# Autodesk Inventor assembly: 044-DPK
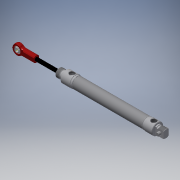
[picture p0: Inventor's stored thumbnail of the model, 180x180]
Saved by Autodesk Inventor 2019.4 (Build 234330000, 330)
## iProperties
Category: PARTsolutions
Company: BIMBA
Created: 2020-02-04
Part Number: 044-DPK
Catalog Web Link: www.cadenas.de
Description: Original Line Standard Air Cylinders-Standard Air Cylinders
Vendor: BIMBA
Document SubType Name: Assembly
Designer: psadmin
Manufacturer: BIMBA
Mass: 35.6804 g
Surface Area: 306.76 cm^2
Volume: 35.6804 cm^3
Density: 1 g/cm^3
PSOL_IDENT_0: {$CADENAS_DATA\23d-libs\bimba\bimba_brand\bimba_imperial\bimba_full_line\original_line_cylinders\sta
PSOL_IDENT_1: ndard_air_cylinders\standard_air_cylinder_asmtab.prj},322 {VTYP=3D},{STYP=ASSTAB},{NB=044-DPK},{LINA=
PSOL_IDENT_2: 044-DPK},{NN=Original Line Standard Air Cylinders},{DATE=22.01.2020 09:07:35},{GEOMDATE=24.10.2019 0
PSOL_IDENT_3: 9:09:47},{VERSION=},{LINEID=50},{WBVAR=STROKE,ACTING,MNT,DER,NR,BM,CO,OO,VO,M,EE,EEL,K,Q,Y,G,T,HL,B,
PSOL_IDENT_4: H,SER,SR,NT,W,STPT1,STPT2,STPT3,STPT4,MB,PB,PRC,TB,MN},{WBNUMERIC=STROKE,EEL}  {NB=044-DPK},{LINA=04
PSOL_IDENT_5: 4-DPK},{KT=DUMMY},{PN=044-DPK},{PNC=044-DPK},{PNA=(NO ACCESSORIES)},{DASH=-},{BORE1=0.75000000},{BOR
PSOL_IDENT_6: E=3/4\" (04)},{BOREPN=04},{STROKE=4.000},{STROKEALG=[0.011:50/0.001]},{STROKE1=4.000},{ACTING=D},{AC
PSOL_IDENT_7: TINGALG= '' , 'Single Acting' , 'R' , 'Reverse Single Acting (R)' , 'D' , 'Double Acting (D)' },{ACT
PSOL_IDENT_8: INGPN=D},{MNT=P},{MNTALG= '' , 'Front Nose Mounting' , 'P' , 'Rear Pivot Mounting (P)' , 'XP' , 'Dou
PSOL_IDENT_9: ble End or Pivot Mounting (XP)' , 'X' , 'Double End Mounting (X)' , 'BF' , 'Front Block Mounting (BF
PSOL_IDENT_10: )' , 'BR' , 'Rear Block Mounting for Vertical Positioning (BR)' , 'BFT' , 'Front Block Trunnion Moun
PSOL_IDENT_11: ting (BFT)' , 'BRT' , 'Rear Block Trunnion Mounting (BRT)' },{TYPE=},{MNTPN=P},{DER=},{DERALG= '' , '
PSOL_IDENT_12: N/A' },{NR=},{NRALG= '' , 'N/A' },{NRPN=},{BM=},{BMALG= '' , 'N/A' },{BMPN=},{CO=},{COALG= '' , 'N/A'
PSOL_IDENT_13: },{OO=},{OOALG= '', 'N/A' },{OOPN=},{VO=Z},{VOALG= 'Z' , 'N/A' },{VOPN=},{OOVOPN=},{M=},{MALG= '', '
PSOL_IDENT_14: Without Magnet', 'M', 'With Magnet' },{EE=},{EEL=0.000},{EEMAX=46.0000},{EEALG= '', 'Without Extra E
PSOL_IDENT_15: xtension', 'EE', 'With Extra Extension' },{EELALG=0},{EEPN=},{EEPN1=0.000},{K=K},{KALG= '', 'Standar
PSOL_IDENT_16: d' , 'K' , 'Ports Rotated 90deg K' },{KPN=K},{Q=},{QALG= '' , 'N/A' },{QPN=},{Y=},{YALG= '' , 'Witho
PSOL_IDENT_17: ut Pivot Bushing' , 'Y' , 'With Pivot Bushing' },{YPN=},{YCON=},{F=},{FALG= '', 'Non-Coated (Standar
PSOL_IDENT_18: d)', 'F', 'Molycoated' },{FPN=},{G=},{GPN=},{GPN99=},{T=},{TALG= '' , 'Standard -20° to 200°F (-29°
PSOL_IDENT_19: to 95°C)' , 'N' , 'Low Temperature' , 'V' , 'High Temperature' },{NPN=},{VPN=},{HL=},{HLALG= '' , 'W
PSOL_IDENT_20: ithout Low Pressure Hydraulic' , 'HL' , 'With Low Pressure Hydraulic' },{B=},{BALG= '', 'W/out Bumpe
PSOL_IDENT_21: rs' , 'B' , 'W/ Bumpers' },{BPN=},{H=},{HALG= '', 'N/A' },{HPN=},{SER=},{SERALG= '' , 'Without Sprin
PSOL_IDENT_22: g Extend/Return' , 'JS' , 'With Spring Return' , 'JR' , 'With Spring Extend' },{SR=C},{SRALG= 'C' , '
PSOL_IDENT_23: Standard Blackened Carbon Steel' , 'SR' , 'Stainless Steel [SR]' },{SRPN=},{SRCON=1},{NT=},{NTPN=},{
PSOL_IDENT_24: W=},{WALG= '' , 'Without Wiper' , 'W' , 'With Wiper' },{WPN=},{E=},{EALG= '' , 'Standard Seals/Lube'
PSOL_IDENT_25: , 'E' , 'Non-Lube Seals/Lube' },{EPN=},{ST=},{STALG= '' , 'N/A' },{STPT1=},{STPT1ALG= '' , 'N/A' },
PSOL_IDENT_26: {STPT2=},{STPT2ALG= '' , 'N/A' },{STPT3=},{STPT3ALG= '' , 'N/A' },{STPT4=},{STPT4ALG= '' , 'N/A' },{
PSOL_IDENT_27: STPN=},{MB=},{MBALG= '' , 'N/A' },{MBPN=},{MBPNALL=},{MBPNALLREAR=},{PB=},{PBALG= '' , 'Without Pivo
PSOL_IDENT_28: t Bracket' , 'D-167' , 'D-167' },{PBPN=},{PBPNALL=D-167},{PRC=},{PRCALG= '' , 'W/out Pivot Rod Clevi
PSOL_IDENT_29: s' , 'F,D-166-3' , 'D-166-3 (front)' },{PRCPN=},{PRCPNALL=D-166-3},{TB=},{TBALG= '' , 'N/A' },{TBPN=
PSOL_IDENT_30: },{TBPNALL=},{MN=},{MNALG= '' , 'Without Mounting Nut' , 'F,D-9' , 'D-9 (front)' , 'R,D-9' , 'D-9 (r
PSOL_IDENT_31: ear)', '2x,D-9' , 'D-9 (front & rear)' },{MNPN=},{MNCONF=},{MNCONR=},{TLEN=5.2555},{FRAC=22.7500},{R
PSOL_IDENT_32: GCON=},{RGDACCON=R},{RHCON=P},{RHCON1=P},{RHCONON=1},{RHACCON=},{FNUTCON=0},{RNUTCON=0},{FNUTPN=D-9}
PSOL_IDENT_33: ,{RNUTPN=D-9},{FNUTTRANS=0.0000},{RNUTTRANS=0.0000},{VHOLECON=0},{A1=1.5940},{A1N=0.8750},{A1P=1.594
PSOL_IDENT_34: 0},{A1B=1.5940},{A4=0.2525},{A4N=0.3130},{A4P=0.2525},{A5=0.0300},{A1H=1.594},{A1NH=0.5310},{A1PH=1.
PSOL_IDENT_35: 5940},{A1BH=1.0940},{A1SH=1.2190},{A2H=0.2190},{A2NH=0.2190},{LENGTH=3.7500},{LENGTH1=3.7500},{LENGT
PSOL_IDENT_36: H2=3.8100},{MUL=4.0000},{MUL11=4.0000},{MUL22=10.76},{MUL33=6.7600},{MUL2=4.0000},{MUL211=4.0000},{M
PSOL_IDENT_37: UL222=2.6900},{MUL233=1.6900},{SSS=8.0000},{RGLEN=1.3715},{RHLEN=1.1230},{SSS1=5.0000},{A13=1.3120},
PSOL_IDENT_38: {DIF=0.0000},{G5=0.6250},{ON=0},{SSADD=0.0000},{BADD=0.0000},{MADD=0.0000},{NVADD=0.0000},{TRACKL=4.
PSOL_IDENT_39: 9655},{TRACKCON=D-74168},{TRIMCON=0},{TRIMCON1=0},{PINCON=D-51},{FSPACE=0.5877},{SPACE=0.0857},{TEXT=
PSOL_IDENT_40: 0.1500},{S1=1.0000},{D1=0.8325},{D1N=0.8050},{D1B=0.8625},{D1P=0.8325},{FA=0.940},{RA=0.9400},{PPATH=
PSOL_IDENT_41: standard_air_cylinder_asmtpl.prj},{MATALGHTML=<b>Standard Original Line:</b><dl><dt>Rod:</dt><dd>- S
PSOL_IDENT_42: tainless Steel</dd><dd>&nbsp;&nbsp;(5/16 9/16 Bores)</dd><dd>- High Strength Carbon Steel</dd><dd>&n
PSOL_IDENT_43: bsp;&nbsp;(3/4 3 Bore)</dd><dd>- Stainless Steel</dd><dd>&nbsp;&nbsp;(X style DXP/DX/DXDE)</dd><dt>B
PSOL_IDENT_44: earings:</dt><dd>- Sintered Bronze</dd><dt>Body:</dt><dd>- 304 Stainless Steel</dd><dt>End Caps:</dt
PSOL_IDENT_45: ><dd>- Aluminum</dd><dt>Seals:</dt><dd>- Buna N</dd></dl>},{ASSCFGPRA=04DP},{MBPNA=},{MNPNA=},{PRCPN
PSOL_IDENT_46: A=},{ASSOPTACC=STPT4},{A=7.75},{HADD=0.0000},{WFL=0.25},{QADD=0.000},{QADD1=0.440},{TEST=4.0000},{MN
PSOL_IDENT_47: TB=},{STDNUTF=0},{STDNUTR=0},{STRK2D=0},{X2D=2},{STROKESW=4.000},{EESW=0.000},{FCD=0},{BCD=0},{RCD=0
PSOL_IDENT_48: },{CUSTADD=3.000},{FT=1/4-28 UNF-2A},{FT1=1/4-28 UNF-2A},{FT2=5/8-18 UNF-2A},{PORT=1/8 NPT},{FT11=1/
PSOL_IDENT_49: 2-20 UNF-2A},{FT12=5/8-18 UNF-2A},{B1=}
NN: Original Line Standard Air Cylinders
NT: Threaded (Standard)
NB: 044-DPK
NBSYN: $PNC.
LINA: 044-DPK
PN: 044-DPK
PNA: (NO ACCESSORIES)
BORE: 3/4" (04)
STROKE: 4
ACTING: Double Acting (D)
MNT: Rear Pivot Mounting (P)
DER: N/A
NR: N/A
BM: N/A
CO: N/A
OO: N/A
VO: N/A
M: Without Magnet
EE: Without Extra Extension
EEL: 0
K: Ports Rotated 90deg K
Q: N/A
Y: Without Pivot Bushing
G: Standard Lube
T: Standard -20° to 200°F (-29° to 95°C)
HL: Without Low Pressure Hydraulic
B: W/out Bumpers
H: N/A
SER: Without Spring Extend/Return
SR: Standard Blackened Carbon Steel
W: Without Wiper
STPT1: N/A
STPT2: N/A
STPT3: N/A
STPT4: N/A
MB: N/A
PB: Without Pivot Bracket
PRC: W/out Pivot Rod Clevis
TB: N/A
MN: Without Mounting Nut
A: 7.75
SUPPLIER: BIMBA
ARTICLENO: 044-DPK
BOMINFO: 044-DPK
CREATOR: CADENAS GmbH
Title: 044-DPK
Author: Cadenas PARTsolutions
Comments: Standard Air Cylinders
## Documents named in this file (8)
- T:\EIT\2020 Infinite Recharge\2020 ROBOT\COMMON PARTS\AIR CYLINDERS\044-DPK\AIS2018\044-DPK.iam
- T:\EIT\2020 Infinite Recharge\2020 ROBOT\COMMON PARTS\AIR CYLINDERS\044-DPK\AIS2018\044-DPCK0000000_0_dummy.ipt
- T:\EIT\2020 Infinite Recharge\2020 ROBOT\COMMON PARTS\AIR CYLINDERS\044-DPK\AIS2018\04RK000-0_rod_guide.ipt
- T:\EIT\2020 Infinite Recharge\2020 ROBOT\COMMON PARTS\AIR CYLINDERS\044-DPK\AIS2018\04R-5_25550C.ipt
- T:\EIT\2020 Infinite Recharge\2020 ROBOT\COMMON PARTS\AIR CYLINDERS\044-DPK\AIS2018\04P0K000_rear_head.ipt
- T:\EIT\2020 Infinite Recharge\2020 ROBOT\COMMON PARTS\AIR CYLINDERS\044-DPK\AIS2018\D-51.ipt
- T:\EIT\2020 Infinite Recharge\2020 ROBOT\COMMON PARTS\AIR CYLINDERS\044-DPK\AIS2018\C-044-DP0000_rod.ipt
- T:\EIT\2020 Infinite Recharge\2020 ROBOT\COMMON PARTS\AIR CYLINDERS\TieRod End\60685K321_PTFE-LINED ALUMINUM BALL JOINT ROD END.ipt
## Components (7 placed, 7 different names)
1. 044-DPCK0000000_0_dummy:1
2. 04RK000-0_rod_guide:1 — Insert:1
3. 04R-5_25550C:1
4. 04P0K000_rear_head:1 — Angle:1
5. D-51:1
6. C-044-DP0000_rod:1 — Insert:1, Insert:2
7. 60685K321_PTFE-LINED ALUMINUM BALL JOINT ROD END:1 — Insert:2, Angle:1
## Relationships (3: Insert 2, Angle 1)
- Insert:1: 04RK000-0_rod_guide:1 ↔ C-044-DP0000_rod:1
- Insert:2: C-044-DP0000_rod:1 ↔ 60685K321_PTFE-LINED ALUMINUM BALL JOINT ROD END:1
- Angle:1 (0 deg): 04P0K000_rear_head:1 ↔ 60685K321_PTFE-LINED ALUMINUM BALL JOINT ROD END:1
